# Autodesk Inventor assembly: Polycarb main conv
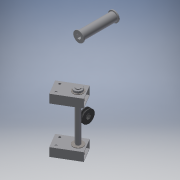
[picture p0: Inventor's stored thumbnail of the model, 180x180]
Saved by Autodesk Inventor 2018 (Build 220112000, 112)
## iProperties
Created: 2020-01-27
Part Number: Polycarb main conv
Document SubType Name: Assembly
Designer: Burni
Author: Burni
## Documents named in this file (7)
- H:\GitHub\2020CAD\Tyler's Ball Storage\Polycarb half main conv.iam
- H:\GitHub\2020CAD\Tyler's Ball Storage\Hex shaft\Shooter hex shaft.ipt
- H:\GitHub\2020CAD\Tyler's Ball Storage\1x2 hexshaft mount.ipt
- H:\GitHub\2020CAD\Tyler's Ball Storage\Other parts\am-2986 FR8ZZ Hex Bearing.ipt
- H:\GitHub\2020CAD\Tyler's Ball Storage\Other parts\Clamping_Shaft_Collar_-_1_2_Hex_ID_217-2737.ipt
- \\studenthome\students\S-4008082\GitHub\2020CAD\Tyler's Ball Storage\Other parts\Polycord conveyor.ipt
- \\studenthome\students\S-4008082\GitHub\2020CAD\Tyler's Ball Storage\Other parts\WCP-0096 Rev1.ipt
## Components (11 placed, 6 different names)
1. Shooter hex shaft:1 — Mate:10, Mate:11, Mate:12, Mate:13, Mate:14, Mate:15, Flush:6, Mate:27, Mate:28, Mate:30, Mate:31
2. 1x2 hexshaft mount:1 — Mate:1, Mate:2, Mate:3, Mate:5, Flush:4, Flush:5, Mate:21
3. 1x2 hexshaft mount:2 — Mate:6, Mate:7, Mate:8, Mate:9, Flush:4, Flush:5, Mate:21, Flush:6
4. am-2986 FR8ZZ Hex Bearing:1 — Mate:7, Mate:8, Mate:12, Mate:13
5. am-2986 FR8ZZ Hex Bearing:2 — Mate:6, Mate:9, Mate:10, Mate:11, Mate:32
6. am-2986 FR8ZZ Hex Bearing:3 — Mate:1, Mate:2, Flush:2, Mate:14, Mate:15
7. am-2986 FR8ZZ Hex Bearing:4 — Mate:3, Mate:5, Flush:2, Mate:29
8. Clamping_Shaft_Collar_-_1_2_Hex_ID_217-2737:1 — Mate:27, Mate:28, Mate:29
9. Clamping_Shaft_Collar_-_1_2_Hex_ID_217-2737:2 — Mate:30, Mate:31, Mate:32
10. Polycord conveyor:1
11. WCP-0096 Rev1:1
## Relationships (25: Mate 21, Flush 4)
- Mate:1: 1x2 hexshaft mount:1 ↔ am-2986 FR8ZZ Hex Bearing:3
- Mate:2: 1x2 hexshaft mount:1 ↔ am-2986 FR8ZZ Hex Bearing:3
- Mate:3: 1x2 hexshaft mount:1 ↔ am-2986 FR8ZZ Hex Bearing:4
- Mate:5: 1x2 hexshaft mount:1 ↔ am-2986 FR8ZZ Hex Bearing:4
- Mate:6: 1x2 hexshaft mount:2 ↔ am-2986 FR8ZZ Hex Bearing:2
- Mate:7: 1x2 hexshaft mount:2 ↔ am-2986 FR8ZZ Hex Bearing:1
- Mate:8: 1x2 hexshaft mount:2 ↔ am-2986 FR8ZZ Hex Bearing:1
- Mate:9: 1x2 hexshaft mount:2 ↔ am-2986 FR8ZZ Hex Bearing:2
- Mate:10: Shooter hex shaft:1 ↔ am-2986 FR8ZZ Hex Bearing:2
- Mate:11: Shooter hex shaft:1 ↔ am-2986 FR8ZZ Hex Bearing:2
- Mate:12: Shooter hex shaft:1 ↔ am-2986 FR8ZZ Hex Bearing:1
- Mate:13: Shooter hex shaft:1 ↔ am-2986 FR8ZZ Hex Bearing:1
- Flush:2: am-2986 FR8ZZ Hex Bearing:3 ↔ am-2986 FR8ZZ Hex Bearing:4
- Mate:14: Shooter hex shaft:1 ↔ am-2986 FR8ZZ Hex Bearing:3
- Mate:15: Shooter hex shaft:1 ↔ am-2986 FR8ZZ Hex Bearing:3
- Flush:4: 1x2 hexshaft mount:1 ↔ 1x2 hexshaft mount:2
- Flush:5: 1x2 hexshaft mount:1 ↔ 1x2 hexshaft mount:2
- Mate:21 (114.3 mm): 1x2 hexshaft mount:1 ↔ 1x2 hexshaft mount:2
- Flush:6 (9.525 mm): Shooter hex shaft:1 ↔ 1x2 hexshaft mount:2
- Mate:27: Shooter hex shaft:1 ↔ Clamping_Shaft_Collar_-_1_2_Hex_ID_217-2737:1
- Mate:28: Shooter hex shaft:1 ↔ Clamping_Shaft_Collar_-_1_2_Hex_ID_217-2737:1
- Mate:29: am-2986 FR8ZZ Hex Bearing:4 ↔ Clamping_Shaft_Collar_-_1_2_Hex_ID_217-2737:1
- Mate:30: Shooter hex shaft:1 ↔ Clamping_Shaft_Collar_-_1_2_Hex_ID_217-2737:2
- Mate:31: Shooter hex shaft:1 ↔ Clamping_Shaft_Collar_-_1_2_Hex_ID_217-2737:2
- Mate:32: am-2986 FR8ZZ Hex Bearing:2 ↔ Clamping_Shaft_Collar_-_1_2_Hex_ID_217-2737:2
